# Autodesk Inventor assembly: LegLinksAssembly
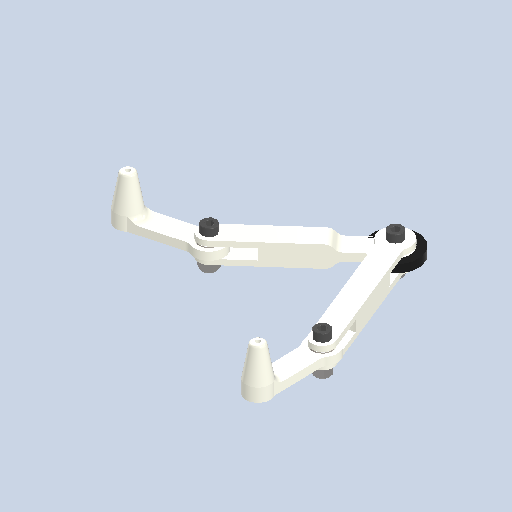
[picture p0: Inventor's stored thumbnail of the model, 512x512]
Saved by Autodesk Inventor 2022 (Build 260153000, 153)
## iProperties
Created: 2021-11-22
Part Number: LegLinksAssembly
Document SubType Name: Assembly
Designer: JK
Mass: 16.0555 g
Surface Area: 94.4419 cm^2
Volume: 9.48605 cm^3
Author: JK
## Documents named in this file (9)
- C:\Users\JK\Documents\Inventor\N20 Leg Actuator\N20-Leg-Actuator\CADfiles\LegLinksAssembly.iam
- C:\Users\JK\Documents\Inventor\N20 Leg Actuator\N20-Leg-Actuator\CADfiles\LinkA SB.ipt
- C:\Users\JK\Documents\Inventor\N20 Leg Actuator\N20-Leg-Actuator\CADfiles\LinkB SB.ipt
- C:\Users\JK\Documents\Inventor\N20 Leg Actuator\N20-Leg-Actuator\CADfiles\LinkC SB.ipt
- C:\Users\JK\Documents\Inventor\N20 Leg Actuator\N20-Leg-Actuator\CADfiles\Rubberfoot.ipt
- C:\Users\JK\Documents\Inventor\N20 Leg Actuator\N20-Leg-Actuator\CADfiles\M3 Locknut.ipt
- C:\Users\JK\Documents\Inventor\N20 Leg Actuator\N20-Leg-Actuator\CADfiles\683zz.ipt
- C:\Users\JK\Documents\Inventor\N20 Leg Actuator\N20-Leg-Actuator\CADfiles\M3x12SocketBolt.ipt
- C:\Users\JK\Documents\Inventor\N20 Leg Actuator\N20-Leg-Actuator\CADfiles\LinkA SB B.ipt
## Components (14 placed, 8 different names)
1. LinkA SB:1 — Coincidencia:23
2. LinkA SB B:1
3. LinkC SB:1 — Coincidencia:21
4. Rubberfoot:1
5. M3 Locknut:1
6. M3 Locknut:2 — Coincidencia:20
7. M3 Locknut:3 — Coincidencia:22
8. 683zz:1
9. 683zz:2
10. 683zz:3
11. M3x12SocketBolt:1
12. M3x12SocketBolt:2 — Coincidencia:18, Coincidencia:19, Coincidencia:20
13. M3x12SocketBolt:3 — Coincidencia:17
14. LinkB SB:2 — Coincidencia:17, Coincidencia:18, Coincidencia:19, Coincidencia:21, Coincidencia:22, Coincidencia:23
## Relationships (27: Mate 17, Flush 9, Angle 1)
- [Flush]: LinkA SB:1 ↔ LinkA SB B:1
- [Mate]: LinkC SB:1 ↔ Rubberfoot:1
- [Flush]: M3 Locknut:1 ↔ M3 Locknut:2
- [Flush]: M3 Locknut:2 ↔ M3 Locknut:3
- [Flush]: LinkC SB:1 ↔ Rubberfoot:1
- [Mate]: LinkA SB:1 ↔ 683zz:1
- [Flush]: LinkA SB:1 ↔ 683zz:1
- [Mate]: LinkA SB B:1 ↔ 683zz:2
- [Flush]: LinkA SB B:1 ↔ 683zz:2
- [Mate]: LinkA SB B:1 ↔ M3x12SocketBolt:1
- [Mate]: LinkC SB:1 ↔ M3x12SocketBolt:3
- [Flush]: M3x12SocketBolt:2 ↔ M3x12SocketBolt:3
- [Mate]: LinkA SB B:1 ↔ LinkC SB:1
- [Mate]: LinkA SB:1 ↔ M3x12SocketBolt:2
- [Flush]: M3x12SocketBolt:1 ↔ M3x12SocketBolt:2
- [Mate]: M3 Locknut:1 ↔ M3x12SocketBolt:1
- [Mate]: LinkC SB:1 ↔ 683zz:3
- [Flush]: LinkC SB:1 ↔ 683zz:3
- [Mate]: M3 Locknut:3 ↔ M3x12SocketBolt:3
- [Angle] (180 deg): LinkC SB:1 ↔ Rubberfoot:1
- Coincidencia:17 [Mate]: M3x12SocketBolt:3 ↔ LinkB SB:2
- Coincidencia:18 [Mate]: M3x12SocketBolt:2 ↔ LinkB SB:2
- Coincidencia:19 [Mate]: M3x12SocketBolt:2 ↔ LinkB SB:2
- Coincidencia:20 [Mate]: M3 Locknut:2 ↔ M3x12SocketBolt:2
- Coincidencia:21 [Mate]: LinkC SB:1 ↔ LinkB SB:2
- Coincidencia:22 [Mate]: M3 Locknut:3 ↔ LinkB SB:2
- Coincidencia:23 [Mate]: LinkA SB:1 ↔ LinkB SB:2
